# Autodesk Inventor assembly: Actuator 1.6
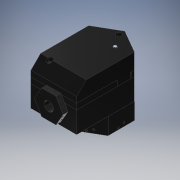
[picture p0: Inventor's stored thumbnail of the model, 180x180]
Saved by Autodesk Inventor 2017 SP1 (Build 210196100, 196)
## iProperties
Created: 2019-09-19
Part Number: Actuator 1.6
Document SubType Name: Assembly
Designer: Dell
Author: Dell
## Documents named in this file (14)
- C:\Users\Zach\Documents\GitHub\tr2\Actuator 1.6\Actuator 1.6.iam
- C:\Users\Zach\Documents\GitHub\tr2\Actuator 1.6\AC01.ipt
- C:\Users\Zach\Documents\GitHub\tr2\Actuator 1.6\AC02.ipt
- C:\Users\Zach\Documents\GitHub\tr2\Actuator 1.6\AC03.ipt
- C:\Users\Zach\Documents\GitHub\tr2\Actuator 1.6\AC05.ipt
- C:\Users\Zach\Documents\GitHub\tr2\Actuator 1.6\Slewing.iam
- C:\Users\Zach\Documents\GitHub\tr2\Actuator 1.6\TSINY TS-42GZ495.ipt
- C:\Users\Zach\Documents\GitHub\tr2\Actuator 1.6\Slip Ring.ipt
- C:\Users\Zach\Documents\GitHub\tr2\Actuator 1.6\8mm Mounting Hub.ipt
- C:\Users\Zach\Documents\GitHub\tr2\Actuator 1.6\Series Elastic Gearbox\Series Elastic Gearbox.iam
- C:\Users\Zach\Documents\GitHub\tr2\Actuator 1.6\Actuator 1.6\Design Accelerator\Spur Gears1.iam
- C:\Users\Zach\Documents\GitHub\tr2\Actuator 1.6\AEAT-6012.ipt
- C:\Users\Zach\Documents\GitHub\tr2\Actuator 1.6\Actuator 1.6\Design Accelerator\Spur Gears2.iam
- C:\Users\Zach\Desktop\AC06.ipt
## Components (14 placed, 12 different names)
1. AC01:1 — Mate:3, Mate:4, Mate:5, Mate:9, Mate:11, Mate:19, Flush:1
2. AC02:1 — Mate:9, Mate:11, Mate:14, Mate:15, Mate:16, Mate:17, Mate:18, Mate:19, Mate:27, Mate:42, Mate:43, Mate:44, Mate:45, Mate:62
3. AC03:1 — Mate:16, Mate:17, Mate:18
4. AC05:1 — Mate:6, Mate:7, Mate:8, Mate:23, Mate:24, Mate:25, Mate:29, Mate:30, Mate:31
5. Slewing:1 [sub-assembly] — Mate:3, Mate:4, Mate:5, Mate:6, Mate:7, Mate:8
6. TSINY TS-42GZ495:1 — Mate:14, Mate:15, Mate:26, Mate:27, Mate:28
7. Slip Ring:2 — Mate:23, Mate:24, Mate:25
8. 8mm Mounting Hub:1 — Mate:26, Mate:28, Mate:36, Mate:37, Mate:64
9. Series Elastic Gearbox:1 [sub-assembly] — Mate:29, Mate:30, Mate:31, Mate:59, Mate:60, Mate:63, Mate:65, Mate:66, Mate:67
10. Spur Gears:1 [sub-assembly] — Mate:36, Mate:37, Mate:64, Mate:65, Mate:66, Mate:67, Rotation:1
11. AEAT-6012:1 — Mate:42, Mate:43, Mate:61
12. AEAT-6012:2 — Mate:44, Mate:45, Mate:68
13. Spur Gears:2 [sub-assembly] — Mate:59, Mate:60, Mate:61, Mate:62, Mate:63
14. AC06:1 — Mate:68, Flush:1, Rotation:1
## Relationships (41: Mate 39, Flush 1, RelateRotation 1)
- Mate:3: AC01:1 ↔ Slewing:1
- Mate:4: AC01:1 ↔ Slewing:1
- Mate:5: AC01:1 ↔ Slewing:1
- Mate:6: AC05:1 ↔ Slewing:1
- Mate:7: AC05:1 ↔ Slewing:1
- Mate:8: AC05:1 ↔ Slewing:1
- Mate:9: AC01:1 ↔ AC02:1
- Mate:11: AC01:1 ↔ AC02:1
- Mate:14: AC02:1 ↔ TSINY TS-42GZ495:1
- Mate:15: AC02:1 ↔ TSINY TS-42GZ495:1
- Mate:16: AC02:1 ↔ AC03:1
- Mate:17: AC02:1 ↔ AC03:1
- Mate:18: AC02:1 ↔ AC03:1
- Mate:19: AC01:1 ↔ AC02:1
- Mate:23: AC05:1 ↔ Slip Ring:2
- Mate:24 (5 mm): AC05:1 ↔ Slip Ring:2
- Mate:25: AC05:1 ↔ Slip Ring:2
- Mate:26: TSINY TS-42GZ495:1 ↔ 8mm Mounting Hub:1
- Mate:27: AC02:1 ↔ TSINY TS-42GZ495:1
- Mate:28 (3 mm): TSINY TS-42GZ495:1 ↔ 8mm Mounting Hub:1
- Mate:29: AC05:1 ↔ Series Elastic Gearbox:1
- Mate:30: AC05:1 ↔ Series Elastic Gearbox:1
- Mate:31: AC05:1 ↔ Series Elastic Gearbox:1
- Mate:36: 8mm Mounting Hub:1 ↔ Spur Gears:1
- Mate:37: 8mm Mounting Hub:1 ↔ Spur Gears:1
- Mate:42: AC02:1 ↔ AEAT-6012:1
- Mate:43: AC02:1 ↔ AEAT-6012:1
- Mate:44: AC02:1 ↔ AEAT-6012:2
- Mate:45: AC02:1 ↔ AEAT-6012:2
- Mate:59: Series Elastic Gearbox:1 ↔ Spur Gears:2
- Mate:60: Series Elastic Gearbox:1 ↔ Spur Gears:2
- Mate:61: AEAT-6012:1 ↔ Spur Gears:2
- Mate:62: AC02:1 ↔ Spur Gears:2
- Mate:63: Series Elastic Gearbox:1 ↔ Spur Gears:2
- Mate:64: 8mm Mounting Hub:1 ↔ Spur Gears:1
- Mate:65: Series Elastic Gearbox:1 ↔ Spur Gears:1
- Mate:66: Series Elastic Gearbox:1 ↔ Spur Gears:1
- Mate:67: Series Elastic Gearbox:1 ↔ Spur Gears:1
- Mate:68: AEAT-6012:2 ↔ AC06:1
- Flush:1: AC01:1 ↔ AC06:1
- Rotation:1 [RelateRotation] (1 ul): Spur Gears:1 ↔ AC06:1
